# Autodesk Inventor assembly: 1x1 tube
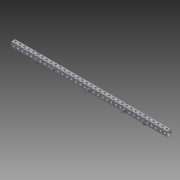
[picture p0: Inventor's stored thumbnail of the model, 180x180]
Saved by Autodesk Inventor 2014 SP1 (Build 180222100, 222)
## iProperties
Created: 2014-03-20
Part Number: 1x1 tube
Document SubType Name: Assembly
Designer: Ryan
Author: Ryan
## Documents named in this file (6)
- C:\Users\Ryan\Desktop\sw\toss up 5th A bot\drive\1x1 tube.iam
- C:\Users\Ryan\Desktop\sw\lib\Aperture VEX CAD Library\Metal\L Bar\1 x 35.ipt
- C:\Users\Ryan\Desktop\sw\lib\Aperture VEX CAD Library\Hardware\8-32\8-32_.875.ipt
- C:\Users\Ryan\Desktop\sw\lib\Aperture VEX CAD Library\Spacers\thin\SPACER-0320-0500.ipt
- C:\Users\Ryan\Desktop\sw\lib\Aperture VEX CAD Library\Hardware\8-32\8-32 nylock.ipt
- C:\Users\Ryan\Desktop\sw\lib\Aperture VEX CAD Library\Spacers\thin\SPACER-0320-0375.ipt
## Components (17 placed, 5 different names)
1. 1 x 35:1 — Flush:1, Flush:2, Flush:3, Mate:1, Mate:3, Mate:4, Mate:5, Mate:17
2. 1 x 35:2 — Flush:1, Flush:2, Flush:3, Mate:7, Mate:11, Mate:12, Mate:13, Mate:18
3. 8-32 nylock:1 — Mate:6, Mate:7
4. 8-32_.875:1 — Mate:1, Mate:2, Mate:5, Mate:6
5. SPACER-0320-0500:1 — Mate:2, Mate:3, Mate:4
6. 8-32 nylock:3
7. 8-32_.875:3
8. SPACER-0320-0500:2
9. SPACER-0320-0375:1 — Mate:16
10. 8-32 nylock:2 — Mate:18
11. 8-32_.875:2 — Mate:11, Mate:12, Mate:13, Mate:16, Mate:17
12. SPACER-0320-0375:2
13. 8-32 nylock:4
14. 8-32_.875:4
15. SPACER-0320-0375:3
16. 8-32 nylock:5
17. 8-32_.875:5
## Component patterns: (2 elements, first: 8-32 nylock:1 + 8-32_.875:1 + SPACER-0320-0500:1), (3 elements, first: SPACER-0320-0375:1 + 8-32 nylock:2 + 8-32_.875:2)
## Relationships (18: Mate 15, Flush 3)
- Flush:1: 1 x 35:1 ↔ 1 x 35:2
- Flush:2: 1 x 35:1 ↔ 1 x 35:2
- Flush:3: 1 x 35:1 ↔ 1 x 35:2
- Mate:1: 1 x 35:1 ↔ 8-32_.875:1
- Mate:2: 8-32_.875:1 ↔ SPACER-0320-0500:1
- Mate:3: 1 x 35:1 ↔ SPACER-0320-0500:1
- Mate:4 (2.3114 mm): 1 x 35:1 ↔ SPACER-0320-0500:1
- Mate:5 (2.3114 mm): 1 x 35:1 ↔ 8-32_.875:1
- Mate:6: 8-32 nylock:1 ↔ 8-32_.875:1
- Mate:7 (1.1684 mm): 1 x 35:2 ↔ 8-32 nylock:1
- [Mate]: SPACER-0320-0375:1 ↔ 8-32_.875:2
- [Mate]: 8-32 nylock:2 ↔ 8-32_.875:2
- Mate:11 (2.3114 mm): 1 x 35:2 ↔ 8-32_.875:2
- Mate:12 (2.3114 mm): 1 x 35:2 ↔ 8-32_.875:2
- Mate:13 (2.3114 mm): 1 x 35:2 ↔ 8-32_.875:2
- Mate:16 (1.1684 mm): SPACER-0320-0375:1 ↔ 8-32_.875:2
- Mate:17: 1 x 35:1 ↔ 8-32_.875:2
- Mate:18: 1 x 35:2 ↔ 8-32 nylock:2
## Named parameters: q = 2.3114 mm, d10_d8 = 0 mm, d11_d4 = 0 mm
